# Autodesk Inventor assembly: Snow Blower Motor
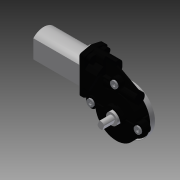
[picture p0: Inventor's stored thumbnail of the model, 180x180]
Saved by Autodesk Inventor 2014 SP1 (Build 180222100, 222)
## iProperties
Created: 2013-01-18
Part Number: Snow Blower Motor
Document SubType Name: Assembly
Designer: actoennies
Mass: 1394.31 g
Surface Area: 470.07 cm^2
Volume: 178.237 cm^3
Density: 7.8228 g/cm^3
Translation Standard: STEP AP203
FileName: AM-2235.STEP
PreProcessor: SolidWorks 2010
PostProcessor: Build: 138, Release: 2013 RTM - Date: Thu 03/01/2012
Sent Units: inch
Uncertainty: 1e-05
Author: actoennies
## Documents named in this file (6)
- C:\Users\Moses\Documents\Inventor\Sally Rebuild\Rebuild Sally\Snow Blower Motor.iam
- C:\Users\Moses\Documents\Inventor\Sally Rebuild\Rebuild Sally\AM-2235 output shaft.ipt
- C:\Users\Moses\Documents\Inventor\Sally Rebuild\Rebuild Sally\AM-2235 gearbox housing.ipt
- C:\Users\Moses\Documents\Inventor\Sally Rebuild\Rebuild Sally\AM-2235 threaded insert.ipt
- C:\Users\Moses\Documents\Inventor\Sally Rebuild\Rebuild Sally\AM-2235 motor.ipt
- C:\Users\Moses\Documents\Inventor\Sally Rebuild\Rebuild Sally\AM-2235 gear cap.ipt
## Components (7 placed, 5 different names)
1. AM-2235 output shaft:1 — Insert:1
2. AM-2235 gearbox housing:1 — Insert:1
3. AM-2235 threaded insert:1
4. AM-2235 motor:1
5. AM-2235 threaded insert:2
6. AM-2235 threaded insert:3
7. AM-2235 gear cap:1
## Relationships (1: Insert 1)
- Insert:1: AM-2235 output shaft:1 ↔ AM-2235 gearbox housing:1
